# Autodesk Inventor assembly: khớp nối mắt trâu lỗ 4mm
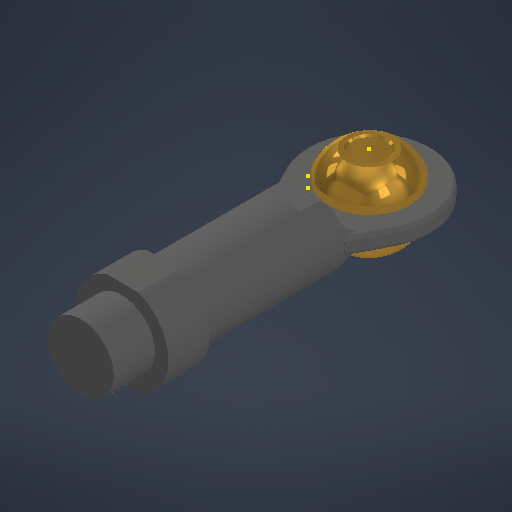
[picture p0: Inventor's stored thumbnail of the model, 512x512]
Saved by Autodesk Inventor 2027.1 (Build 311270010, 270A)
## iProperties
Created: 2026-08-09
Part Number: khớp nối mắt trâu lỗ 4mm
Document SubType Name: Assembly
Designer: MSI
Author: MSI
## Documents named in this file (3)
- C:\Users\MSI\Documents\MECHATRONICS\Tot_nghiep\Do_an_Delta.Robot_Dang_Rui_Bi\Thiết kế\Delta Part\khớp nối mắt trâu lỗ 4mm.iam
- C:\Users\MSI\Documents\MECHATRONICS\Tot_nghiep\Do_an_Delta.Robot_Dang_Rui_Bi\Thiết kế\Delta Part\mắt trâu.ipt
- C:\Users\MSI\Documents\MECHATRONICS\Tot_nghiep\Do_an_Delta.Robot_Dang_Rui_Bi\Thiết kế\Delta Part\vòng bi_dài 35mm.ipt
## Components (2 placed, 2 different names)
1. mắt trâu:1 — Mate:1
2. vòng bi_dài 35mm:1 — Mate:1
## Relationships (1: Mate 1)
- Mate:1: mắt trâu:1 ↔ vòng bi_dài 35mm:1
